# Autodesk Inventor assembly: outerboxassembly
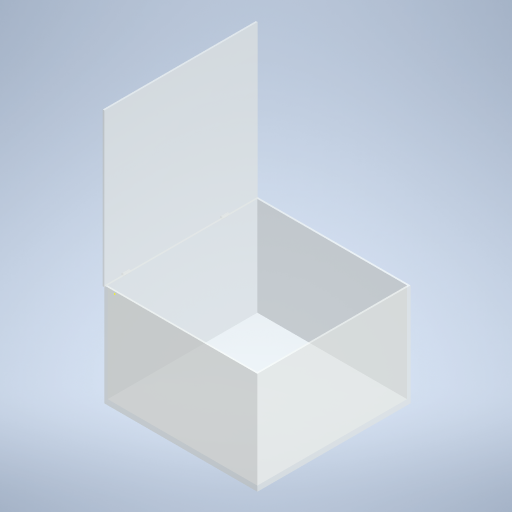
[picture p0: Inventor's stored thumbnail of the model, 512x512]
Saved by Autodesk Inventor 2024 (Build 280153000, 153)
## iProperties
Created: 2023-06-07
Part Number: outerboxassembly
Document SubType Name: Assembly
Designer: badig
Author: badig
## Documents named in this file (4)
- C:\Users\shraa\Downloads\outerboxassembly.iam
- C:\Users\shraa\Downloads\rectangle box.ipt
- C:\Users\shraa\Downloads\rectangle upper portion.ipt
- C:\Users\shraa\Downloads\boxholder.ipt
## Components (4 placed, 3 different names)
1. rectangle box:1 — Mate:1, Mate:3
2. rectangle upper portion:1 — Mate:1, Mate:2
3. boxholder:1 — Mate:2
4. boxholder:2 — Mate:3
## Relationships (3: Mate 3)
- Mate:1: rectangle box:1 ↔ rectangle upper portion:1
- Mate:2: rectangle upper portion:1 ↔ boxholder:1
- Mate:3: rectangle box:1 ↔ boxholder:2
